# Autodesk Inventor assembly: Грубая сборка
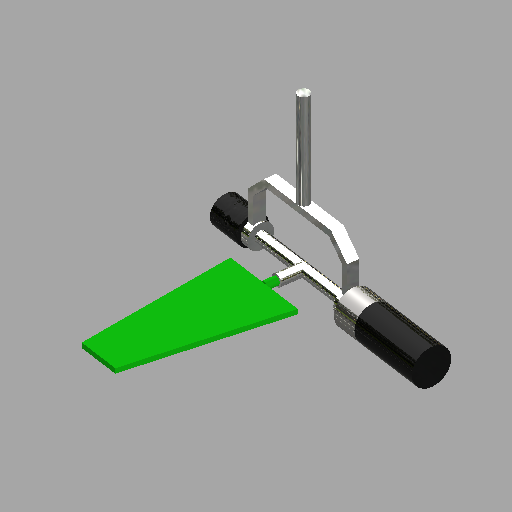
[picture p0: Inventor's stored thumbnail of the model, 512x512]
Saved by Autodesk Inventor 2025 (Build 290162000, 162)
## iProperties
Created: 2024-11-27
Part Number: Грубая сборка
Document SubType Name: Assembly
Designer: Artem Sannikov
Mass: 212.59 g
Surface Area: 220.391 cm^2
Volume: 47.9271 cm^3
Density: 4.43569 g/cm^3
Author: Artem Sannikov
## Documents named in this file (7)
- C:\Users\Artem Sannikov\Desktop\Two_axis_gimbal\3D_модели\Вспомогательные модели\Грубая сборка.iam
- C:\Users\Artem Sannikov\Desktop\Two_axis_gimbal\3D_модели\Вспомогательные модели\Макет_рамки.ipt
- C:\Users\Artem Sannikov\Desktop\Two_axis_gimbal\3D_модели\Вспомогательные модели\Ось_антенны.ipt
- C:\Users\Artem Sannikov\Desktop\Two_axis_gimbal\3D_модели\Вспомогательные модели\Антенна.ipt
- C:\Users\Artem Sannikov\Desktop\Two_axis_gimbal\3D_модели\Вспомогательные модели\Редуктор.ipt
- C:\Users\Artem Sannikov\Desktop\Two_axis_gimbal\3D_модели\Вспомогательные модели\Двигатель.ipt
- C:\Users\Artem Sannikov\Desktop\Two_axis_gimbal\3D_модели\Вспомогательные модели\Энкодер.ipt
## Components (6 placed, 6 different names)
1. Макет_рамки:1 — Совмещение:1, Заподлицо:1, Совмещение:2, Совмещение:3, Заподлицо:2, Угол:1
2. Ось_антенны:1 — Совмещение:1, Заподлицо:1, Совмещение:4, Совмещение:5, Совмещение:6, Совмещение:7, Совмещение:10, Совмещение:11
3. Антенна:1 — Совмещение:4, Совмещение:5, Угол:1
4. Редуктор:1 — Совмещение:6, Совмещение:7, Совмещение:8, Совмещение:9
5. Двигатель:1 — Совмещение:8, Совмещение:9
6. Энкодер:1 — Совмещение:10, Совмещение:11
## Relationships (14: Mate 11, Flush 2, Angle 1)
- Совмещение:1 [Mate]: Макет_рамки:1 ↔ Ось_антенны:1
- Заподлицо:1 [Flush] (-1 mm): Макет_рамки:1 ↔ Ось_антенны:1
- Совмещение:2 [Mate]: Макет_рамки:1
- Совмещение:3 [Mate]: Макет_рамки:1
- Заподлицо:2 [Flush]: Макет_рамки:1
- Совмещение:4 [Mate]: Ось_антенны:1 ↔ Антенна:1
- Совмещение:5 [Mate]: Ось_антенны:1 ↔ Антенна:1
- Совмещение:6 [Mate]: Ось_антенны:1 ↔ Редуктор:1
- Совмещение:7 [Mate]: Ось_антенны:1 ↔ Редуктор:1
- Совмещение:8 [Mate]: Редуктор:1 ↔ Двигатель:1
- Совмещение:9 [Mate]: Редуктор:1 ↔ Двигатель:1
- Совмещение:10 [Mate]: Ось_антенны:1 ↔ Энкодер:1
- Совмещение:11 [Mate]: Ось_антенны:1 ↔ Энкодер:1
- Угол:1 [Angle] (0 deg): Макет_рамки:1 ↔ Антенна:1
